# Autodesk Inventor assembly: gripper manufacturing layout
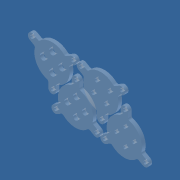
[picture p0: Inventor's stored thumbnail of the model, 180x180]
Saved by Autodesk Inventor 2012 (Build 160160000, 160)
## iProperties
Created: 2013-01-23
Part Number: gripper manufacturing layout
Document SubType Name: Assembly
Designer: Edward
Author: Edward
## Documents named in this file (5)
- C:\Users\Edward\Documents\masters\Mechanical\Gripper\gripper manufacturing layout.iam
- C:\Users\Edward\Documents\masters\Mechanical\Gripper\acrylic gripper plate 2.ipt
- C:\Users\Edward\Documents\masters\Mechanical\Gripper\acrylic gripper plate.ipt
- C:\Users\Edward\Documents\masters\Mechanical\Gripper\acrylic IRB120 plate 2.ipt
- C:\Users\Edward\Documents\masters\Mechanical\Gripper\acrylic IRB120 plate.ipt
## Components (4 placed, 4 different names)
1. acrylic gripper plate 2:1 — Flush:1, Tangent:2, Tangent:3, Angle:2, Tangent:4, Angle:3
2. acrylic gripper plate:1 — Flush:1, Flush:2, Tangent:1, Tangent:3, Angle:1, Angle:2
3. acrylic IRB120 plate 2:1 — Flush:2, Flush:3, Tangent:1, Tangent:2, Angle:1, Tangent:5
4. acrylic IRB120 plate:1 — Flush:3, Tangent:4, Angle:3, Tangent:5
## Relationships (11: Tangent 5, Flush 3, Angle 3)
- Flush:1: acrylic gripper plate 2:1 ↔ acrylic gripper plate:1
- Flush:2: acrylic gripper plate:1 ↔ acrylic IRB120 plate 2:1
- Flush:3: acrylic IRB120 plate 2:1 ↔ acrylic IRB120 plate:1
- Tangent:1 (1.27 mm): acrylic gripper plate:1 ↔ acrylic IRB120 plate 2:1
- Tangent:2 (1.27 mm): acrylic gripper plate 2:1 ↔ acrylic IRB120 plate 2:1
- Tangent:3 (1.27 mm): acrylic gripper plate 2:1 ↔ acrylic gripper plate:1
- Angle:1 (180 deg): acrylic gripper plate:1 ↔ acrylic IRB120 plate 2:1
- Angle:2 (0 deg): acrylic gripper plate 2:1 ↔ acrylic gripper plate:1
- Tangent:4 (1.27 mm): acrylic gripper plate 2:1 ↔ acrylic IRB120 plate:1
- Angle:3 (0 deg): acrylic gripper plate 2:1 ↔ acrylic IRB120 plate:1
- Tangent:5 (1.27 mm): acrylic IRB120 plate 2:1 ↔ acrylic IRB120 plate:1
